# Autodesk Inventor assembly: msl
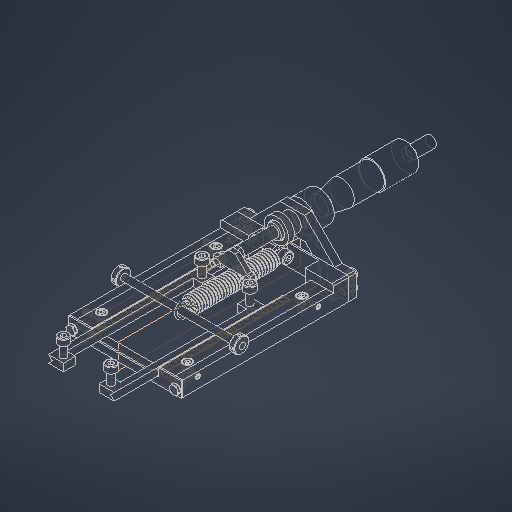
[picture p0: Inventor's stored thumbnail of the model, 512x512]
Saved by Autodesk Inventor 2026.1 (Build 301233020, 233B)
## iProperties
Created: 2025-11-03
Part Number: msl
Document SubType Name: Assembly
Designer: Jan
Author: Jan
## Documents named in this file (23)
- C:\Users\Jan\OneDrive\Pulpit\inventor\MSL\msl.iam
- C:\Users\Jan\OneDrive\Pulpit\inventor\MSL\podstawa.ipt
- C:\Users\Jan\OneDrive\Pulpit\inventor\MSL\GM-150-804.ipt
- C:\Users\Jan\OneDrive\Pulpit\inventor\MSL\K-tor-kulek.ipt
- C:\Users\Jan\OneDrive\Pulpit\inventor\MSL\uchwyt-GM.ipt
- C:\Users\Jan\OneDrive\Pulpit\inventor\MSL\kula_d4mm.ipt
- C:\Users\Jan\OneDrive\Pulpit\inventor\MSL\separator-kul.ipt
- C:\Users\Jan\OneDrive\Pulpit\inventor\MSL\K-tor-kulek-blatu.ipt
- C:\Users\Jan\OneDrive\Pulpit\inventor\MSL\K-tor-kulek-blatu_MIR.ipt
- C:\Users\Jan\OneDrive\Pulpit\inventor\MSL\blat.ipt
- C:\Users\Jan\OneDrive\Pulpit\inventor\MSL\spr-naciagowa.ipt
- C:\Users\Jan\OneDrive\Documents\Inventor\Content Center Files\R2026\en-US\AS 1420\AS 1420 - 1973 - M4 x 30.ipt
- C:\Users\Jan\OneDrive\Pulpit\inventor\MSL\wałek-blatu.ipt
- C:\Users\Jan\OneDrive\Documents\Inventor\Content Center Files\R2026\en-US\CNS 4433\CNS 4433 - M 4.ipt
- C:\Users\Jan\OneDrive\Pulpit\inventor\MSL\stopka.ipt
- C:\Users\Jan\OneDrive\Documents\Inventor\Content Center Files\R2026\en-US\AS 1420\AS 1420 - 1973 - M4 x 12.ipt
- C:\Users\Jan\OneDrive\Documents\Inventor\Content Center Files\R2026\en-US\AS 1421(2)\AS 1421 - M3 x 4 Cup Point.ipt
- C:\Users\Jan\OneDrive\Documents\Inventor\Content Center Files\R2026\en-US\AS 1110\AS 1110 - M3 x 6.ipt
- C:\Users\Jan\OneDrive\Documents\Inventor\Content Center Files\R2026\en-US\AS 1110\AS 1110 - M3 x 12.ipt
- C:\Users\Jan\OneDrive\Documents\Inventor\Content Center Files\R2026\en-US\AS 1420\AS 1420 - 1973 - M3 x 6.ipt
- C:\Users\Jan\OneDrive\Pulpit\inventor\MSL\nakretka-GM.ipt
- C:\Users\Jan\OneDrive\Pulpit\inventor\MSL\oslonka.ipt
- C:\Users\Jan\OneDrive\Pulpit\inventor\MSL\wkladka gumowa.ipt
## Components (70 placed, 22 different names)
1. podstawa:1 — Mate:1, Mate:2, Mate:3, Mate:4, Mate:5, Mate:6, Angle:1, Angle:2, Flush:4, Mate:8, Mate:12, Mate:13, Flush:7, Mate:17, Mate:21, Flush:10, Flush:11, Mate:26, Mate:27, Mate:28, Mate:37, Flush:13, Mate:41, Mate:46, Flush:19, Flush:20, Insert:14, Insert:15, Insert:16, Insert:17
2. GM-150-804:1 — Mate:20, Tangent:6
3. K-tor-kulek:1 — Mate:4, Mate:5, Mate:6, Mate:11, Insert:8, Insert:9, Mate:39, Flush:16, Tangent:10, Tangent:11
4. K-tor-kulek:2 — Mate:1, Mate:2, Mate:3, Tangent:2, Tangent:3, Flush:5, Insert:10, Insert:11, Flush:15
5. uchwyt-GM:1 — Mate:20, Mate:21, Flush:10, Flush:11, Tangent:6, Mate:29, Mate:30, Mate:31, Mate:32, Mate:33, Mate:34, Mate:35, Mate:36, Mate:42, Mate:43
6. separator-kul:1 — Angle:1, Angle:2, Flush:15
7. K-tor-kulek-blatu:1 — Mate:8, Flush:5, Flush:8, Mate:14
8. K-tor-kulek-blatu_MIR:1 — Flush:6, Mate:13, Flush:14, Mate:44
9. blat:1 — Flush:7, Flush:8, Mate:14, Tangent:5, Flush:9, Mate:19, Mate:22, Mate:23, Insert:2, Insert:3, Insert:4, Flush:12, Mate:38, Mate:39, Flush:13, Flush:14, Mate:40, Tangent:9
10. spr-naciagowa:1
11. AS 1420 - Metric M4 x 30:1 — Mate:41
12. wałek-blatu:1 — Tangent:5, Flush:9, Mate:16, Mate:18, Tangent:9
13. CNS 4433 M 4:1 — Mate:16, Mate:17
14. CNS 4433 M 4:2 — Mate:18, Mate:19
15. stopka:1 — Insert:5, Insert:6, Flush:12, Mate:38
16. AS 1420 - Metric M4 x 12:1 — Mate:22, Mate:23
17. AS 1420 - Metric M4 x 12:2 — Insert:2
18. AS 1420 - Metric M4 x 12:3 — Insert:3
19. AS 1420 - Metric M4 x 12:4 — Insert:4, Mate:44
20. AS 1421 Cup Point - Metric M3 x 4 Cup Point:2 — Mate:26
21. AS 1421 Cup Point - Metric M3 x 4 Cup Point:3 — Mate:27
22. AS 1421 Cup Point - Metric M3 x 4 Cup Point:4 — Mate:28
23. AS 1421 Cup Point - Metric M3 x 4 Cup Point:5 — Mate:37
24. AS 1110 - Metric M3 x 12:1 — Mate:29, Mate:30
25. AS 1110 - Metric M3 x 12:2 — Mate:31, Mate:32
26. AS 1110 - Metric M3 x 12:3 — Mate:33, Mate:34
27. AS 1110 - Metric M3 x 12:4 — Mate:35, Mate:36
28. AS 1110 - Metric M3 x 6:1 — Insert:5
29. AS 1110 - Metric M3 x 6:2 — Insert:6, Mate:40
30. AS 1420 - Metric M3 x 6:1 — Insert:8
31. AS 1420 - Metric M3 x 6:2 — Insert:9
32. AS 1420 - Metric M3 x 6:3 — Insert:10
33. AS 1420 - Metric M3 x 6:4 — Insert:11
34. nakretka-GM:1 — Mate:42, Mate:43
35. separator-kul:2 — Flush:16
36. oslonka:2 — Mate:46, Flush:19, Flush:20, Insert:12, Insert:13
37. AS 1110 - Metric M3 x 6:4 — Insert:12
38. AS 1110 - Metric M3 x 6:3 — Insert:13
39. wkladka gumowa:1 — Insert:14
40. wkladka gumowa:2 — Insert:17
41. wkladka gumowa:3 — Insert:16
42. wkladka gumowa:4 — Insert:15
43. kula_d4mm:1 — Tangent:2, Tangent:3
44. kula_d4mm:2
45. kula_d4mm:3
46. kula_d4mm:4
47. kula_d4mm:5
48. kula_d4mm:6
49. kula_d4mm:7
50. kula_d4mm:8
51. kula_d4mm:9
52. kula_d4mm:10
53. kula_d4mm:11
54. kula_d4mm:12
55. kula_d4mm:13
56. kula_d4mm:14
57. kula_d4mm:15 — Tangent:10, Tangent:11
58. kula_d4mm:16
59. kula_d4mm:17
60. kula_d4mm:18
61. kula_d4mm:19
62. kula_d4mm:20
63. kula_d4mm:21
64. kula_d4mm:22
65. kula_d4mm:23
66. kula_d4mm:24
67. kula_d4mm:25
68. kula_d4mm:26
69. kula_d4mm:27
70. kula_d4mm:28
## Component patterns: (14 elements, first: kula_d4mm:1), (14 elements, first: kula_d4mm:15)
## Relationships (78: Mate 39, Flush 15, Insert 15, Tangent 7, Angle 2)
- Mate:1: podstawa:1 ↔ K-tor-kulek:2
- Mate:2: podstawa:1 ↔ K-tor-kulek:2
- Mate:3: podstawa:1 ↔ K-tor-kulek:2
- Mate:4: podstawa:1 ↔ K-tor-kulek:1
- Mate:5: podstawa:1 ↔ K-tor-kulek:1
- Mate:6: podstawa:1 ↔ K-tor-kulek:1
- Tangent:2: K-tor-kulek:2 ↔ kula_d4mm:1
- Tangent:3: K-tor-kulek:2 ↔ kula_d4mm:1
- Angle:1 (0 deg): podstawa:1 ↔ separator-kul:1
- Angle:2 (0 deg): podstawa:1 ↔ separator-kul:1
- Flush:4 (-37.5 mm): podstawa:1
- Mate:8: podstawa:1 ↔ K-tor-kulek-blatu:1
- Flush:5: K-tor-kulek:2 ↔ K-tor-kulek-blatu:1
- Mate:11: K-tor-kulek:1
- Mate:12: podstawa:1
- Flush:6: K-tor-kulek-blatu_MIR:1
- Mate:13: podstawa:1 ↔ K-tor-kulek-blatu_MIR:1
- Flush:7: podstawa:1 ↔ blat:1
- Flush:8: K-tor-kulek-blatu:1 ↔ blat:1
- Mate:14: K-tor-kulek-blatu:1 ↔ blat:1
- Tangent:5: blat:1 ↔ wałek-blatu:1
- Flush:9 (-4 mm): blat:1 ↔ wałek-blatu:1
- Mate:16: wałek-blatu:1 ↔ CNS 4433 M 4:1
- Mate:17: podstawa:1 ↔ CNS 4433 M 4:1
- Mate:18: wałek-blatu:1 ↔ CNS 4433 M 4:2
- Mate:19: blat:1 ↔ CNS 4433 M 4:2
- Mate:20: GM-150-804:1 ↔ uchwyt-GM:1
- Mate:21: podstawa:1 ↔ uchwyt-GM:1
- Flush:10: podstawa:1 ↔ uchwyt-GM:1
- Flush:11: podstawa:1 ↔ uchwyt-GM:1
- Tangent:6: GM-150-804:1 ↔ uchwyt-GM:1
- Mate:22: blat:1 ↔ AS 1420 - Metric M4 x 12:1
- Mate:23: blat:1 ↔ AS 1420 - Metric M4 x 12:1
- Insert:2: blat:1 ↔ AS 1420 - Metric M4 x 12:2
- Insert:3: blat:1 ↔ AS 1420 - Metric M4 x 12:3
- Insert:4: blat:1 ↔ AS 1420 - Metric M4 x 12:4
- Mate:26: podstawa:1 ↔ AS 1421 Cup Point - Metric M3 x 4 Cup Point:2
- Mate:27: podstawa:1 ↔ AS 1421 Cup Point - Metric M3 x 4 Cup Point:3
- Mate:28: podstawa:1 ↔ AS 1421 Cup Point - Metric M3 x 4 Cup Point:4
- Mate:29: uchwyt-GM:1 ↔ AS 1110 - Metric M3 x 12:1
- Mate:30: uchwyt-GM:1 ↔ AS 1110 - Metric M3 x 12:1
- Mate:31: uchwyt-GM:1 ↔ AS 1110 - Metric M3 x 12:2
- Mate:32: uchwyt-GM:1 ↔ AS 1110 - Metric M3 x 12:2
- Mate:33: uchwyt-GM:1 ↔ AS 1110 - Metric M3 x 12:3
- Mate:34: uchwyt-GM:1 ↔ AS 1110 - Metric M3 x 12:3
- Mate:35: uchwyt-GM:1 ↔ AS 1110 - Metric M3 x 12:4
- Mate:36: uchwyt-GM:1 ↔ AS 1110 - Metric M3 x 12:4
- Insert:5: stopka:1 ↔ AS 1110 - Metric M3 x 6:1
- Insert:6: stopka:1 ↔ AS 1110 - Metric M3 x 6:2
- Insert:8: K-tor-kulek:1 ↔ AS 1420 - Metric M3 x 6:1
- Insert:9: K-tor-kulek:1 ↔ AS 1420 - Metric M3 x 6:2
- Insert:10: K-tor-kulek:2 ↔ AS 1420 - Metric M3 x 6:3
- Insert:11: K-tor-kulek:2 ↔ AS 1420 - Metric M3 x 6:4
- Mate:37: podstawa:1 ↔ AS 1421 Cup Point - Metric M3 x 4 Cup Point:5
- Flush:12: blat:1 ↔ stopka:1
- Mate:38: blat:1 ↔ stopka:1
- Mate:39: K-tor-kulek:1 ↔ blat:1
- Flush:13: podstawa:1 ↔ blat:1
- Flush:14: K-tor-kulek-blatu_MIR:1 ↔ blat:1
- Mate:40: blat:1 ↔ AS 1110 - Metric M3 x 6:2
- Mate:41: podstawa:1 ↔ AS 1420 - Metric M4 x 30:1
- Mate:42: uchwyt-GM:1 ↔ nakretka-GM:1
- Mate:43: uchwyt-GM:1 ↔ nakretka-GM:1
- Tangent:9: blat:1 ↔ wałek-blatu:1
- Flush:15: K-tor-kulek:2 ↔ separator-kul:1
- Mate:44: K-tor-kulek-blatu_MIR:1 ↔ AS 1420 - Metric M4 x 12:4
- Flush:16: K-tor-kulek:1 ↔ separator-kul:2
- Tangent:10: K-tor-kulek:1 ↔ kula_d4mm:15
- Tangent:11: K-tor-kulek:1 ↔ kula_d4mm:15
- Mate:46: podstawa:1 ↔ oslonka:2
- Flush:19: podstawa:1 ↔ oslonka:2
- Flush:20: podstawa:1 ↔ oslonka:2
- Insert:12: oslonka:2 ↔ AS 1110 - Metric M3 x 6:4
- Insert:13: oslonka:2 ↔ AS 1110 - Metric M3 x 6:3
- Insert:14: podstawa:1 ↔ wkladka gumowa:1
- Insert:15: podstawa:1 ↔ wkladka gumowa:4
- Insert:16: podstawa:1 ↔ wkladka gumowa:3
- Insert:17: podstawa:1 ↔ wkladka gumowa:2
